# Autodesk Inventor assembly: ASY MSC 900.3 base frame
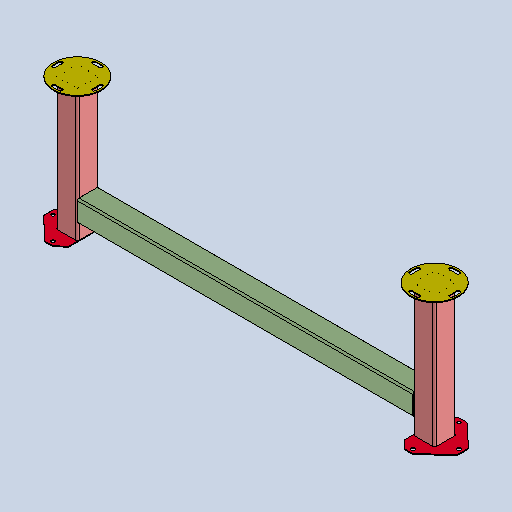
[picture p0: Inventor's stored thumbnail of the model, 512x512]
Saved by Autodesk Inventor 2025 (Build 290162010, 162A)
## iProperties
_SolveAssemblyDoc: Frame Generator Solve Assembly
_Version: 25.0.0
Created: 2024-06-27
Part Number: ASY MSC 900.3 base frame
Document SubType Name: Assembly
Designer: admin
Stock Number: ASY МОО 900.3 базовая рама
Author: admin
## Documents named in this file (6)
- C:\Users\admin\YandexDisk-badmisterfox\домашниий пк\Inventor\Manturovo\Manturovo_Se-clar\Рама основания\ASY MSC 120  base frame.iam
- C:\Users\admin\YandexDisk-badmisterfox\домашниий пк\Inventor\Manturovo\Manturovo_Se-clar\Рама основания\MSC 100 base frame.ipt
- C:\Users\admin\YandexDisk-badmisterfox\домашниий пк\Inventor\Manturovo\Manturovo_Se-clar\Рама основания\ASY MSC 120  base frame\Frame\Frame 1719510697528.iam
- C:\Users\admin\YandexDisk-badmisterfox\домашниий пк\Inventor\Manturovo\Manturovo_Se-clar\Чертеж для парам. рамы.ipt
- C:\Users\admin\YandexDisk-badmisterfox\домашниий пк\Inventor\Manturovo\Manturovo_Se-clar\MSC 126 flange frame.ipt
- C:\Users\admin\YandexDisk-badmisterfox\домашниий пк\Inventor\Manturovo\Manturovo_Se-clar\MSC 127 flange frame heel.ipt
## Components (6 placed, 4 different names)
1. MSC 100 base frame:1 — Mate:2
2. Frame 1719510697528:1 [sub-assembly] — Rigid:1, Flush:2, Rigid:2, Rigid:3, Rigid:4
3. MSC 126 flange frame:1 — Rigid:1
4. MSC 126 flange frame:2 — Rigid:2
5. MSC 127 flange frame heel:1 — Rigid:4
6. MSC 127 flange frame heel:2 — Flush:2, Rigid:3
## Relationships (6: WeldJoint 4, Mate 1, Flush 1)
- Rigid:1 [WeldJoint]: Frame 1719510697528:1 ↔ MSC 126 flange frame:1
- Mate:2: MSC 100 base frame:1
- Flush:2: Frame 1719510697528:1 ↔ MSC 127 flange frame heel:2
- Rigid:2 [WeldJoint]: Frame 1719510697528:1 ↔ MSC 126 flange frame:2
- Rigid:3 [WeldJoint]: Frame 1719510697528:1 ↔ MSC 127 flange frame heel:2
- Rigid:4 [WeldJoint]: Frame 1719510697528:1 ↔ MSC 127 flange frame heel:1
## Named parameters: frame_1 = 334.24956 mm, frame_3 = 2905.4 mm, frame_4 = 4190.97522 mm, frame_5 = 5476.55043 mm, Ширина_рамы = 1400 mm, Отступ_до_ниж_перекладины = 100 mm, Отступ_до_верх_перекладины = 350 mm, Шаг_опор_по_баку = 2000 mm, Движение_рамы_вперед_назад = 270 mm, frame_2 = 1619.82478 mm, frame_6 = 6762.12565 mm
